# Autodesk Inventor assembly: IM_Mold_plate_top.ipt
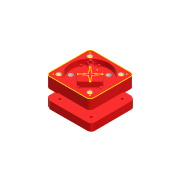
[picture p0: Inventor's stored thumbnail of the model, 180x180]
Saved by Autodesk Inventor 2022 (Build 260153000, 153)
## iProperties
Created: 2023-04-12
Part Number: IM_Mold_plate_top.ipt
Document SubType Name: Assembly
Designer: diederichbenedict
Author: diederichbenedict
## Documents named in this file (5)
- C:\Users\diederichbenedict\Dropbox\Dokumente\Promotion\PROJECTS\Matchboxscope\INVENTOR\RELEASE\Matchboxscope\Workspace\IM_Mold_plate_top.ipt.iam
- C:\Users\diederichbenedict\Dropbox\Dokumente\Promotion\PROJECTS\Matchboxscope\INVENTOR\RELEASE\Matchboxscope\Workspace\IM_Matchboxscope_plate.ipt
- C:\Users\diederichbenedict\Dropbox\Dokumente\Promotion\PROJECTS\Matchboxscope\INVENTOR\RELEASE\Matchboxscope\Workspace\IM_Mold_plate.ipt
- C:\Users\diederichbenedict\Dropbox\Dokumente\Promotion\PROJECTS\Matchboxscope\INVENTOR\RELEASE\Matchboxscope\Workspace\Bauteil1.ipt
- C:\Users\diederichbenedict\Dropbox\Dokumente\Promotion\PROJECTS\Matchboxscope\INVENTOR\RELEASE\Matchboxscope\Workspace\Bauteil2.ipt
## Components (4 placed, 4 different names)
1. IM_Matchboxscope_plate:1 — Fluchtend:1, Fluchtend:2
2. IM_Mold_plate:1 — Fluchtend:1, Fluchtend:2, Passend:1, Passend:2
3. Bauteil1:1 — Passend:1, Passend:2
4. Bauteil2:1
## Relationships (4: Flush 2, Mate 2)
- Fluchtend:1 [Flush]: IM_Matchboxscope_plate:1 ↔ IM_Mold_plate:1
- Fluchtend:2 [Flush]: IM_Matchboxscope_plate:1 ↔ IM_Mold_plate:1
- Passend:1 [Mate]: IM_Mold_plate:1 ↔ Bauteil1:1
- Passend:2 [Mate]: IM_Mold_plate:1 ↔ Bauteil1:1
